# Autodesk Inventor assembly: 1 cell
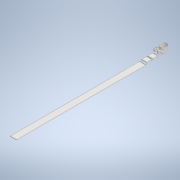
[picture p0: Inventor's stored thumbnail of the model, 180x180]
Saved by Autodesk Inventor 2020 (Build 240168000, 168)
## iProperties
Created: 2019-09-26
Part Number: 1 cell
Document SubType Name: Assembly
Designer: Abbas
Author: Abbas
## Documents named in this file (14)
- D:\Projects\aquaponic\Inventor\1 cell.iam
- D:\Projects\aquaponic\Inventor\fish tank 1.ipt
- D:\Projects\aquaponic\Inventor\swirl filter.ipt
- D:\Projects\aquaponic\Inventor\mineralisation.ipt
- C:\Users\Abbas\Documents\Inventor\Content Center Files\R2020\en-US\ASTM D 2466 90\ASTM D 2466 90 Deg Elbow Socket-Type - Schedule 40 4.ipt
- D:\Projects\aquaponic\Inventor\grow bed.ipt
- D:\Projects\aquaponic\Inventor\dwc.ipt
- D:\Projects\aquaponic\Inventor\ASTM D 1785 Bell-End Pipe 4 - Schedule 40 - 8.ipt
- D:\Projects\aquaponic\Inventor\ASTM D 1785 Pipe 4 - Schedule 40 - 50.ipt
- C:\Users\Abbas\Documents\Inventor\Content Center Files\R2020\en-US\JIS B 2301 ii - CI\JIS B 2301 Bushing Pattern ii - Class I 4 x 3.ipt
- C:\Users\Abbas\Documents\Inventor\Content Center Files\R2020\en-US\JIS B 2301 ii - CI\JIS B 2301 Bushing Pattern ii - Class I 6 x 5.ipt
- C:\Users\Abbas\Documents\Inventor\Content Center Files\R2020\en-US\ISO 3633 45 (10)\ISO 3633 90 Deg Bend with Single Socket for Cemented Type Joints DN110.ipt
- C:\Users\Abbas\Documents\Inventor\Content Center Files\R2020\en-US\ISO 3633 45 (10)\ISO 3633 90 Deg Bend with Single Socket for Cemented Type Joints DN90.ipt
- D:\Projects\aquaponic\Inventor\ISO 4422-2 Pipe 225 x 5.5 PN 6.3 - 250.ipt
## Components (17 placed, 13 different names)
1. fish tank 1:1
2. swirl filter:1 — Insert:1, Angle:1
3. mineralisation:1 — Mate:1, Insert:5, Insert:6, Insert:7, Angle:1
4. ASTM D 2466 90 Deg Elbow Socket-Type - Schedule 40 4:1 — Insert:1, Insert:2
5. grow bed:1
6. grow bed:2
7. dwc:1 — Insert:4
8. ASTM D 1785 Bell-End Pipe 4 - Schedule 40 - 8:1 — Insert:2, Insert:3
9. ASTM D 1785 Pipe 4 - Schedule 40 - 50:1 — Insert:3, Mate:1
10. JIS B 2301 Bushing Pattern ii - Class I 4 x 3:1
11. JIS B 2301 Bushing Pattern ii - Class I 6 x 5:1 — Insert:4
12. ISO 3633 90 Deg Bend with Single Socket for Cemented Type Joints DN110:1 — Insert:5
13. ISO 3633 90 Deg Bend with Single Socket for Cemented Type Joints DN90:1 — Insert:6
14. ISO 3633 90 Deg Bend with Single Socket for Cemented Type Joints DN90:2
15. ISO 3633 90 Deg Bend with Single Socket for Cemented Type Joints DN90:3 — Insert:7
16. ISO 4422-2 Pipe 225 x 5.5 PN 6.3 - 250:1
17. ISO 3633 90 Deg Bend with Single Socket for Cemented Type Joints DN90:4
## Relationships (9: Insert 7, Mate 1, Angle 1)
- Insert:1: swirl filter:1 ↔ ASTM D 2466 90 Deg Elbow Socket-Type - Schedule 40 4:1
- Insert:2 (-20 mm): ASTM D 2466 90 Deg Elbow Socket-Type - Schedule 40 4:1 ↔ ASTM D 1785 Bell-End Pipe 4 - Schedule 40 - 8:1
- Insert:3: ASTM D 1785 Bell-End Pipe 4 - Schedule 40 - 8:1 ↔ ASTM D 1785 Pipe 4 - Schedule 40 - 50:1
- Mate:1: mineralisation:1 ↔ ASTM D 1785 Pipe 4 - Schedule 40 - 50:1
- Insert:4 (-30 mm): dwc:1 ↔ JIS B 2301 Bushing Pattern ii - Class I 6 x 5:1
- Insert:5: mineralisation:1 ↔ ISO 3633 90 Deg Bend with Single Socket for Cemented Type Joints DN110:1
- Insert:6: mineralisation:1 ↔ ISO 3633 90 Deg Bend with Single Socket for Cemented Type Joints DN90:1
- Insert:7: mineralisation:1 ↔ ISO 3633 90 Deg Bend with Single Socket for Cemented Type Joints DN90:3
- Angle:1 (0 deg): swirl filter:1 ↔ mineralisation:1
